# Autodesk Inventor assembly: walektymrazedlugi
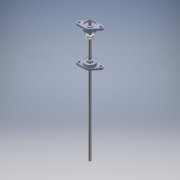
[picture p0: Inventor's stored thumbnail of the model, 180x180]
Saved by Autodesk Inventor 2019 (Build 230136000, 136)
## iProperties
Created: 2020-08-21
Part Number: walektymrazedlugi
Material: Ogólny
Document SubType Name: Assembly
Designer: barto
Author: barto
## Documents named in this file (4)
- C:\Users\estee\OneDrive\Pulpit\estere\1\MUM\wogoleNajnowszyGit\Mechanika\Moduł obrotu RET Estera\prawieKoncowka\walektymrazedlugi.iam
- C:\Users\estee\OneDrive\Pulpit\estere\1\MUM\wogoleNajnowszyGit\Mechanika\Moduł obrotu RET Estera\prawieKoncowka\UCFL-201.ipt
- C:\Users\estee\OneDrive\Pulpit\estere\1\MUM\wogoleNajnowszyGit\Mechanika\Moduł obrotu RET Estera\prawieKoncowka\DIN 471 - 12 x 1(1).ipt
- C:\Users\estee\OneDrive\Pulpit\estere\1\MUM\wogoleNajnowszyGit\Mechanika\Moduł obrotu RET Estera\prawieKoncowka\ModulDuzegoKolaKrotki.iam
## Components (5 placed, 3 different names)
1. ModulDuzegoKolaKrotki:1 [sub-assembly] — Zestawiające:23, Zestawiające:30
2. DIN 471 > 9mm <= 300mm 12 x 1:1 — Zestawiające:23
3. UCFL-201:1
4. UCFL-201:2 — Zestawiające:31
5. DIN 471 > 9mm <= 300mm 12 x 1:2 — Zestawiające:30, Zestawiające:31
## Relationships (3: Mate 3)
- Zestawiające:23 [Mate]: ModulDuzegoKolaKrotki:1 ↔ DIN 471 > 9mm <= 300mm 12 x 1:1
- Zestawiające:30 [Mate]: ModulDuzegoKolaKrotki:1 ↔ DIN 471 > 9mm <= 300mm 12 x 1:2
- Zestawiające:31 [Mate]: UCFL-201:2 ↔ DIN 471 > 9mm <= 300mm 12 x 1:2
## Named parameters: sa_0 = 10000, sa_1 = 0, sa_2 = 0
note: some values were not read from the file. Shown as the stored number, unit unknown: "sa_0", "sa_1", "sa_2".
